# Autodesk Inventor assembly: Traction Wheel full 4in
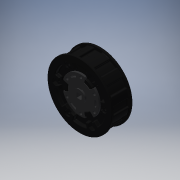
[picture p0: Inventor's stored thumbnail of the model, 180x180]
Saved by Autodesk Inventor 2016 (Build 200138000, 138)
## iProperties
Created: 2019-01-03
Part Number: Traction Wheel full 4in
Document SubType Name: Assembly
Designer: Afnan
Author: Afnan
## Documents named in this file (4)
- D:\New Laptop\(1) New Laptop\AFNAN ALI flashdrive backup\VEXPARTS\Vex parts\VEXPRO\Wheels\Traction\Traction Wheel full 4in.iam
- D:\New Laptop\(1) New Laptop\AFNAN ALI flashdrive backup\VEXPARTS\Vex parts\VEXPRO\Wheels\Traction\4_Traction_Wheel_-_1_Wide_217-2588.ipt
- D:\New Laptop\(1) New Laptop\AFNAN ALI flashdrive backup\VEXPARTS\Vex parts\VEXPRO\Wheels\Wheel Hub.ipt
- D:\New Laptop\(1) New Laptop\AFNAN ALI flashdrive backup\VEXPARTS\Vex parts\VEXPRO\Wheels\Hex to Square 0.25in.ipt
## Components (5 placed, 3 different names)
1. 4_Traction_Wheel_-_1_Wide_217-2588:1 — Mate:1, Mate:2, Mate:3, Mate:4, Mate:5, Mate:6
2. Wheel Hub:1 — Mate:4, Mate:5, Mate:6, Mate:7, Mate:8, Mate:9
3. Wheel Hub:2 — Mate:1, Mate:2, Mate:3, Mate:10
4. Hex to Square 0.25in:1 — Mate:7, Mate:8, Mate:9, Mate:11, Mate:12
5. Hex to Square 0.25in:2 — Mate:10, Mate:11, Mate:12
## Relationships (12: Mate 12)
- Mate:1: 4_Traction_Wheel_-_1_Wide_217-2588:1 ↔ Wheel Hub:2
- Mate:2: 4_Traction_Wheel_-_1_Wide_217-2588:1 ↔ Wheel Hub:2
- Mate:3: 4_Traction_Wheel_-_1_Wide_217-2588:1 ↔ Wheel Hub:2
- Mate:4: 4_Traction_Wheel_-_1_Wide_217-2588:1 ↔ Wheel Hub:1
- Mate:5: 4_Traction_Wheel_-_1_Wide_217-2588:1 ↔ Wheel Hub:1
- Mate:6: 4_Traction_Wheel_-_1_Wide_217-2588:1 ↔ Wheel Hub:1
- Mate:7: Wheel Hub:1 ↔ Hex to Square 0.25in:1
- Mate:8: Wheel Hub:1 ↔ Hex to Square 0.25in:1
- Mate:9: Wheel Hub:1 ↔ Hex to Square 0.25in:1
- Mate:10: Wheel Hub:2 ↔ Hex to Square 0.25in:2
- Mate:11: Hex to Square 0.25in:1 ↔ Hex to Square 0.25in:2
- Mate:12: Hex to Square 0.25in:1 ↔ Hex to Square 0.25in:2
